# Autodesk Inventor assembly: Montagem2
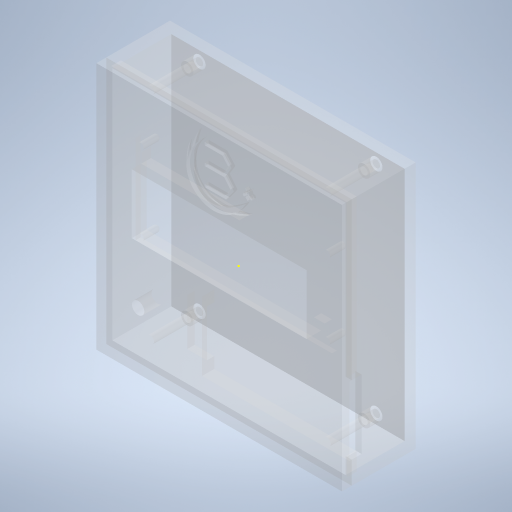
[picture p0: Inventor's stored thumbnail of the model, 512x512]
Saved by Autodesk Inventor 2023 (Build 270158000, 158)
## iProperties
Created: 2022-12-13
Part Number: Montagem2
Document SubType Name: Assembly
Designer: Inteli
Author: Inteli
## Documents named in this file (3)
- C:\Users\Inteli\Documents\GitHub\Projeto3\src\Inventor - Protótipo da CAse\Montagem\Montagem2.iam
- C:\Users\Inteli\Documents\GitHub\Projeto3\src\Inventor - Protótipo da CAse\Peças\Base ESP.ipt
- C:\Users\Inteli\Documents\GitHub\Projeto3\src\Inventor - Protótipo da CAse\Peças\base_frontal_esp.ipt
## Components (2 placed, 2 different names)
1. Base ESP:1 — Coincidente:1, Coincidente:2, Coincidente:3
2. base_frontal_esp:1 — Coincidente:1, Coincidente:2, Coincidente:3
## Relationships (3: Mate 3)
- Coincidente:1 [Mate]: Base ESP:1 ↔ base_frontal_esp:1
- Coincidente:2 [Mate]: Base ESP:1 ↔ base_frontal_esp:1
- Coincidente:3 [Mate]: Base ESP:1 ↔ base_frontal_esp:1
